# Autodesk Inventor assembly: Claw
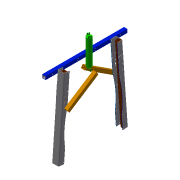
[picture p0: Inventor's stored thumbnail of the model, 180x180]
Saved by Autodesk Inventor 2015 (Build 190159000, 159)
## iProperties
Created: 2015-01-13
Part Number: Claw
Document SubType Name: Assembly
Designer: Collin_2
Author: Collin_2
## Documents named in this file (9)
- C:\Users\Tanner\Documents\GitHub\FIRST-Team-1719-CAD-Team\2015 Robot CAD\Devices\Elevator and Claw\Claw\Claw.iam
- C:\Users\Tanner\Documents\Claw\clawBase.ipt
- C:\Users\Tanner\Documents\GitHub\FIRST-Team-1719-CAD-Team\2015 Robot CAD\Devices\Elevator and Claw\Claw\PC3.5-P1.ipt
- C:\Users\Tanner\Documents\GitHub\FIRST-Team-1719-CAD-Team\2015 Robot CAD\Devices\Elevator and Claw\Claw\PC3.5-ROD.ipt
- C:\Users\Tanner\Documents\Claw\clawRTOP-v2.ipt
- C:\Users\Tanner\Documents\Claw\clawRBOTTOM-v2.ipt
- C:\Users\Tanner\Documents\Claw\ClawArmBeam.ipt
- C:\Users\Tanner\Documents\GitHub\FIRST-Team-1719-CAD-Team\2015 Robot CAD\Devices\Elevator and Claw\Claw\Yarm.ipt
- C:\Users\Tanner\Documents\Inventor\ElevatorCAD\Clawplate.ipt
## Components (13 placed, 8 different names)
1. clawBase:1 — Mate:18, Mate:19, Mate:20, Mate:21, Tangent:1, Tangent:2, Flush:1
2. PC3.5-P1:1 — Mate:15, Mate:16, Tangent:1, Tangent:2, Flush:1
3. PC3.5-ROD:1 — Mate:15, Mate:16, Angle:1, Mate:37
4. clawRTOP-v2:1 — Mate:20, Mate:21, Mate:26, Mate:27, Angle:1, Mate:38, Mate:43, Insert:4
5. clawRTOP-v2:2 — Mate:23, Mate:24, Mate:31, Mate:35, Mate:45, Flush:5, Insert:3
6. clawRBOTTOM-v2:1 — Mate:18, Mate:19, Mate:23, Mate:24, Mate:41, Mate:45, Insert:2, Flush:7
7. clawRBOTTOM-v2:2 — Mate:26, Mate:27, Mate:43, Flush:4, Mate:47, Flush:6, Insert:1, Mate:48, Mate:49
8. ClawArmBeam:1 — Mate:31, Mate:41, Flush:5
9. ClawArmBeam:2 — Flush:4, Mate:48, Mate:49
10. Yarm:1 — Mate:35, Mate:37, Mate:40, Insert:3
11. Yarm:2 — Mate:38, Mate:40, Insert:4
12. Clawplate:1 — Mate:47, Flush:6, Insert:1
13. Clawplate:2 — Insert:2, Flush:7
## Relationships (33: Mate 21, Flush 5, Insert 4, Tangent 2, Angle 1)
- Mate:15: PC3.5-P1:1 ↔ PC3.5-ROD:1
- Mate:16: PC3.5-P1:1 ↔ PC3.5-ROD:1
- Mate:18: clawBase:1 ↔ clawRBOTTOM-v2:1
- Mate:19: clawBase:1 ↔ clawRBOTTOM-v2:1
- Mate:20: clawBase:1 ↔ clawRTOP-v2:1
- Mate:21: clawBase:1 ↔ clawRTOP-v2:1
- Mate:23: clawRTOP-v2:2 ↔ clawRBOTTOM-v2:1
- Mate:24: clawRTOP-v2:2 ↔ clawRBOTTOM-v2:1
- Mate:26: clawRTOP-v2:1 ↔ clawRBOTTOM-v2:2
- Mate:27: clawRTOP-v2:1 ↔ clawRBOTTOM-v2:2
- Angle:1 (0 deg): PC3.5-ROD:1 ↔ clawRTOP-v2:1
- Mate:31: clawRTOP-v2:2 ↔ ClawArmBeam:1
- Mate:35: clawRTOP-v2:2 ↔ Yarm:1
- Mate:37: PC3.5-ROD:1 ↔ Yarm:1
- Mate:38: clawRTOP-v2:1 ↔ Yarm:2
- Mate:40: Yarm:1 ↔ Yarm:2
- Tangent:1: clawBase:1 ↔ PC3.5-P1:1
- Tangent:2 (285.75 mm): clawBase:1 ↔ PC3.5-P1:1
- Flush:1 (-114.3 mm): clawBase:1 ↔ PC3.5-P1:1
- Mate:41: clawRBOTTOM-v2:1 ↔ ClawArmBeam:1
- Mate:43: clawRTOP-v2:1 ↔ clawRBOTTOM-v2:2
- Mate:45: clawRTOP-v2:2 ↔ clawRBOTTOM-v2:1
- Flush:4: clawRBOTTOM-v2:2 ↔ ClawArmBeam:2
- Flush:5: clawRTOP-v2:2 ↔ ClawArmBeam:1
- Mate:47: clawRBOTTOM-v2:2 ↔ Clawplate:1
- Flush:6: clawRBOTTOM-v2:2 ↔ Clawplate:1
- Insert:1: clawRBOTTOM-v2:2 ↔ Clawplate:1
- Insert:2: clawRBOTTOM-v2:1 ↔ Clawplate:2
- Flush:7: clawRBOTTOM-v2:1 ↔ Clawplate:2
- Mate:48: clawRBOTTOM-v2:2 ↔ ClawArmBeam:2
- Mate:49: clawRBOTTOM-v2:2 ↔ ClawArmBeam:2
- Insert:3: clawRTOP-v2:2 ↔ Yarm:1
- Insert:4: clawRTOP-v2:1 ↔ Yarm:2
